# Autodesk Inventor assembly: intakemotorbearing_MIR
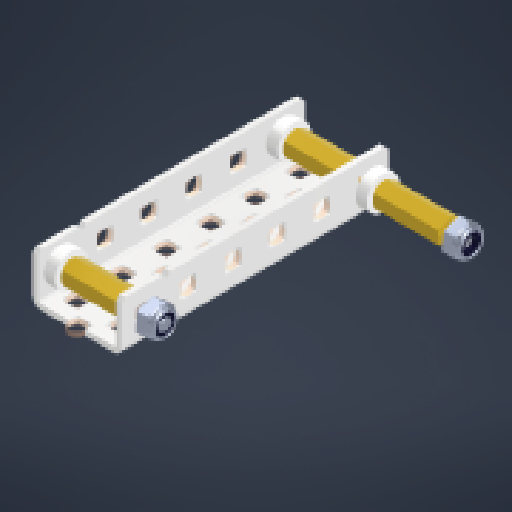
[picture p0: Inventor's stored thumbnail of the model, 512x512]
Saved by Autodesk Inventor 2023 (Build 270158000, 158)
## iProperties
Created: 2023-08-10
Part Number: intakemotorbearing_MIR
Document SubType Name: Assembly
Designer: srbel
Author: srbel
## Documents named in this file (9)
- C:\CAD\OverUnderCAD\Drive\intakemotorbearing_MIR.iam
- C:\CAD\OverUnderCAD\VEX-CAD-Inventor-1.4.0\Motion\Spacers\Spacer Nylon .313 OD\NSpacer .313 OD x .125.ipt
- C:\CAD\OverUnderCAD\VEX-CAD-Inventor-1.4.0\Motion\Spacers\Spacer Nylon .313 OD.ipt
- C:\CAD\OverUnderCAD\VEX-CAD-Inventor-1.4.0\Structure\Standoff\Standoff .75.ipt
- C:\CAD\OverUnderCAD\VEX-CAD-Inventor-1.4.0\Structure\Standoff.ipt
- C:\CAD\OverUnderCAD\VEX-CAD-Inventor-1.4.0\Structure\Hardware\Nut Thin Nylock_MIR7_MIR1_MIR1_MIR_MIR.ipt
- C:\CAD\OverUnderCAD\VEX-CAD-Inventor-1.4.0\Structure\Hardware\Screw Steel - Star.ipt
- C:\CAD\OverUnderCAD\VEX-CAD-Inventor-1.4.0\Structure\C Channel\Aluminum 1x2x1\Alu C 1x2x1x6_MIR3.ipt
- C:\CAD\OverUnderCAD\VEX-CAD-Inventor-1.4.0\Structure\Hardware\Screw Steel - Star\SScrew Star Threaded 1.250.ipt
## Components (10 placed, 5 different names)
1. NSpacer .313 OD x .125:1 — Insert:3, Insert:11
2. Standoff .75:1 — Insert:3
3. NSpacer .313 OD x .125:2 — Insert:3, Insert:14
4. Standoff .75:2 — Insert:3
5. NSpacer .313 OD x .125:3 — Insert:5, Insert:12
6. Standoff .75:3 — Insert:5, Insert:9
7. Nut Thin Nylock_MIR7_MIR1_MIR1_MIR_MIR:1 — Insert:9
8. Nut Thin Nylock_MIR7_MIR1_MIR1_MIR_MIR:2 — Insert:15
9. Alu C 1x2x1x6_MIR3:1 — Insert:15, Insert:14, Insert:12, Insert:11, Insert:16
10. SScrew Star Threaded 1.250:2 — Insert:16
## Relationships (9: Insert 9)
- Insert:3: NSpacer .313 OD x .125:1 ↔ Standoff .75:1
- Insert:3: NSpacer .313 OD x .125:2 ↔ Standoff .75:2
- Insert:5: NSpacer .313 OD x .125:3 ↔ Standoff .75:3
- Insert:9 (1.5875 mm): Standoff .75:3 ↔ Nut Thin Nylock_MIR7_MIR1_MIR1_MIR_MIR:1
- Insert:15 (1.5875 mm): Nut Thin Nylock_MIR7_MIR1_MIR1_MIR_MIR:2 ↔ Alu C 1x2x1x6_MIR3:1
- Insert:14: NSpacer .313 OD x .125:2 ↔ Alu C 1x2x1x6_MIR3:1
- Insert:12 (1.5875 mm): NSpacer .313 OD x .125:3 ↔ Alu C 1x2x1x6_MIR3:1
- Insert:11: NSpacer .313 OD x .125:1 ↔ Alu C 1x2x1x6_MIR3:1
- Insert:16: Alu C 1x2x1x6_MIR3:1 ↔ SScrew Star Threaded 1.250:2
